# Autodesk Inventor assembly: AssemblyFullPrinter
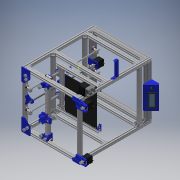
[picture p0: Inventor's stored thumbnail of the model, 180x180]
Saved by Autodesk Inventor 2018 (Build 220112000, 112)
## iProperties
Created: 2017-10-01
Part Number: AssemblyFullPrinter
Document SubType Name: Assembly
Designer: Jurjen
Author: Jurjen
## Documents named in this file (51)
- C:\Users\Jurjen\Documents\3D Printer\coreXY\Mechanical\AssemblyFullPrinter.iam
- C:\Users\Jurjen\Documents\3D Printer\coreXY\Mechanical\2020-350mm.ipt
- C:\Users\Jurjen\Documents\3D Printer\coreXY\Mechanical\2020-500mm.ipt
- C:\Users\Jurjen\Documents\3D Printer\coreXY\Mechanical\2020-corner-bracket.ipt
- C:\Users\Jurjen\Documents\3D Printer\coreXY\Mechanical\heated-bed.ipt
- C:\Users\Jurjen\Documents\3D Printer\coreXY\Mechanical\T8-lead-screw.ipt
- C:\Users\Jurjen\Documents\3D Printer\coreXY\Mechanical\motedis\GT2-Pulley-20-Teeth-5mm-Bore.ipt
- C:\Users\Jurjen\Documents\3D Printer\coreXY\Mechanical\motedis\Gt20.ipt
- C:\Users\Jurjen\Documents\3D Printer\coreXY\Mechanical\motedis\shaft-couple-flex.ipt
- C:\Users\Jurjen\Documents\3D Printer\coreXY\Mechanical\motedis\Motedis-SH8.ipt
- C:\Users\Jurjen\Documents\3D Printer\coreXY\Mechanical\rod-8mm.ipt
- C:\Users\Jurjen\Documents\3D Printer\coreXY\Mechanical\2020-290mm.ipt
- C:\Users\Jurjen\Documents\3D Printer\coreXY\Mechanical\2020-240mm.ipt
- C:\Users\Jurjen\Documents\3D Printer\coreXY\Mechanical\T8x2mm lead screw.ipt
- C:\Users\Jurjen\Documents\3D Printer\coreXY\Mechanical\OldhamCouplerBottom.ipt
- C:\Users\Jurjen\Documents\3D Printer\coreXY\Mechanical\OldhamCouplerMiddle.ipt
- C:\Users\Jurjen\Documents\3D Printer\coreXY\Mechanical\OldhamCouplerTop.ipt
- C:\Users\Jurjen\Documents\3D Printer\coreXY\Mechanical\M5-nut.ipt
- C:\Users\Jurjen\Documents\3D Printer\coreXY\Mechanical\bracket-GT2-left.ipt
- C:\Users\Jurjen\Documents\3D Printer\coreXY\Mechanical\M5x30mm.ipt
- C:\Users\Jurjen\Documents\3D Printer\coreXY\Mechanical\mount-heated-bed.ipt
- C:\Users\Jurjen\Documents\3D Printer\coreXY\Mechanical\bracket-GT2-right.ipt
- C:\Users\Jurjen\Documents\3D Printer\coreXY\Mechanical\spool-holder.ipt
- C:\Users\Jurjen\Documents\3D Printer\coreXY\Mechanical\nema-17.ipt
- C:\Users\Jurjen\Documents\3D Printer\coreXY\Mechanical\nema17-mount-left.ipt
- C:\Users\Jurjen\Documents\3D Printer\coreXY\Mechanical\nema17-mount-right.ipt
- C:\Users\Jurjen\Documents\3D Printer\coreXY\Mechanical\LMF8LUU.ipt
- C:\Users\Jurjen\Documents\3D Printer\coreXY\Mechanical\holder-LMF8LUU-z-axis.ipt
- C:\Users\Jurjen\Documents\3D Printer\coreXY\Mechanical\MGN-12-rail.ipt
- C:\Users\Jurjen\Documents\3D Printer\coreXY\Mechanical\2020-320mm.ipt
- C:\Users\Jurjen\Documents\3D Printer\coreXY\Mechanical\x-carriage-2020.ipt
- C:\Users\Jurjen\Documents\3D Printer\coreXY\Mechanical\X-connector-left.ipt
- C:\Users\Jurjen\Documents\3D Printer\coreXY\Mechanical\X-connector-right.ipt
- C:\Users\Jurjen\Documents\3D Printer\coreXY\Mechanical\MGN-12-H-carriage.ipt
- C:\Users\Jurjen\Documents\3D Printer\coreXY\Mechanical\ED3V6.ipt
- C:\Users\Jurjen\Documents\3D Printer\coreXY\Mechanical\x-carriage.ipt
- C:\Users\Jurjen\Documents\3D Printer\coreXY\Mechanical\x-carriage-holder.ipt
- C:\Users\Jurjen\Documents\3D Printer\coreXY\Mechanical\holder-GT2-x-carriage-left.ipt
- C:\Users\Jurjen\Documents\3D Printer\coreXY\Mechanical\M5x35mm-crosshead.ipt
- C:\Users\Jurjen\Documents\3D Printer\coreXY\Mechanical\extruder\e3d titan.iam
- C:\Users\Jurjen\Documents\3D Printer\coreXY\Mechanical\mount-extruder.ipt
- C:\Users\Jurjen\Documents\3D Printer\coreXY\Mechanical\NylonSpacerM5x5mm.ipt
- C:\Users\Jurjen\Documents\3D Printer\coreXY\Mechanical\holder-GT2-x-carriage-right.ipt
- C:\Users\Jurjen\Documents\3D Printer\coreXY\Mechanical\holder-bearing-z-axis.ipt
- C:\Users\Jurjen\Documents\3D Printer\coreXY\Mechanical\2040-350mm.ipt
- C:\Users\Jurjen\Documents\3D Printer\coreXY\Mechanical\nema17-mount-bottom-z-axis-v2.ipt
- C:\Users\Jurjen\Documents\3D Printer\coreXY\Mechanical\ramps-1.4 2004-LCD.ipt
- C:\Users\Jurjen\Documents\3D Printer\coreXY\Mechanical\holder-LCD-screen.ipt
- C:\Users\Jurjen\Documents\3D Printer\coreXY\Mechanical\spring-25mm.ipt
- C:\Users\Jurjen\Documents\3D Printer\coreXY\Mechanical\M3x40mm.ipt
- C:\Users\Jurjen\Documents\3D Printer\coreXY\Mechanical\2040-360mm.ipt
## Components (158 placed, 50 different names)
1. 2020-500mm:1 — Mate:1, Flush:2, Flush:14, Mate:85, Flush:37, Mate:90, Mate:92, Mate:93, Mate:94, Mate:131, Mate:132, Mate:163, Mate:165, Mate:166, Mate:168, Mate:287, Mate:288, Flush:54, Mate:359, Mate:360, Mate:434, Flush:78, Mate:459, Mate:471, Mate:472, Mate:473, Flush:92, Mate:552, Flush:107, Mate:573, Flush:112, Mate:584, Mate:595
2. 2020-500mm:2 — Mate:2, Flush:1, Flush:13, Flush:14, Mate:75, Mate:77, Mate:79, Mate:80, Mate:133, Mate:135, Mate:151, Mate:152, Mate:154, Mate:156, Mate:362, Mate:439, Mate:455, Mate:530, Flush:93, Mate:563, Flush:109, Flush:110, Flush:113, Mate:574, Mate:590, Mate:592
3. 2020-500mm:3 — Mate:8, Flush:12, Flush:13, Flush:15, Mate:82, Mate:83, Mate:86, Flush:39, Mate:136, Mate:138, Mate:149, Mate:150, Flush:67, Mate:367, Flush:82, Mate:456, Mate:501, Flush:85, Flush:86, Mate:516, Mate:517, Mate:522, Mate:523, Mate:562, Mate:585, Mate:591, Mate:593, Mate:594
4. 2020-500mm:4 — Mate:7, Flush:15, Flush:27, Mate:142, Mate:144, Mate:157, Mate:158, Mate:160, Mate:162, Mate:354, Flush:65, Mate:447, Mate:450, Mate:510, Mate:519, Mate:520, Mate:551, Flush:105, Mate:553, Flush:106, Mate:575, Flush:114, Mate:582, Mate:583, Mate:596
5. 2020-corner-bracket:38 — Mate:515, Mate:516, Mate:517
6. 2020-320mm:3 — Mate:353, Mate:354, Mate:355, Mate:356, Flush:65, Flush:66, Mate:357, Mate:358, Mate:368, Mate:369, Mate:373, Mate:374, Mate:388, Flush:73, Mate:446, Mate:448, Mate:460, Mate:461
7. 2020-320mm:4 — Flush:67, Mate:362, Mate:363, Mate:364, Flush:68, Mate:366, Flush:69, Mate:371, Mate:372, Mate:385, Mate:386, Mate:387, Flush:72, Mate:453, Mate:454, Mate:457, Mate:458
8. 2020-350mm:1 — Mate:1, Mate:2, Flush:1, Flush:2, Mate:19, Mate:23, Mate:76, Mate:95, Mate:294, Mate:303, Mate:304, Mate:307, Mate:308, Flush:66, Flush:68
9. 2020-350mm:4 — Mate:7, Mate:8, Flush:12, Mate:16, Mate:26, Flush:27, Mate:60, Mate:61, Mate:64, Mate:65, Mate:66, Mate:67, Mate:239, Mate:277, Mate:279, Flush:53, Mate:337, Flush:70, Mate:449, Mate:452, Mate:497, Mate:498, Mate:499, Mate:500, Flush:88, Flush:89, Mate:515
10. 2020-corner-bracket:1 — Mate:16, Mate:356, Mate:452
11. 2020-corner-bracket:2 — Mate:23, Mate:363, Mate:364
12. 2020-corner-bracket:3 — Mate:19, Mate:357, Mate:358
13. 2020-corner-bracket:4 — Mate:26, Mate:385, Mate:386
14. 2020-corner-bracket:10 — Mate:75, Mate:76, Mate:77
15. 2020-corner-bracket:13 — Mate:93, Mate:94, Mate:95, Mate:359
16. 2020-corner-bracket:33 — Mate:449, Mate:450
17. 2020-corner-bracket:34 — Mate:446, Mate:447, Mate:448
18. 2020-corner-bracket:35 — Mate:453, Mate:454, Mate:455
19. 2020-corner-bracket:36 — Mate:456, Mate:457, Mate:458
20. 2020-corner-bracket:37 — Mate:459, Mate:460, Mate:461
21. 2040-360mm:1 — Mate:552, Mate:553, Flush:106, Flush:107, Mate:554, Mate:555, Mate:558, Mate:559, Flush:108, Mate:572
22. 2040-360mm:2 — Mate:562, Mate:563, Flush:109, Flush:110, Mate:564, Mate:565, Mate:567, Flush:111, Mate:571
23. ramps-1.4 2004-LCD:1 — Flush:96, Mate:535, Mate:536
24. holder-LCD-screen:1 — Mate:534, Flush:95, Flush:96, Mate:535, Mate:536
25. 2040-350mm:1 — Mate:501, Flush:85, Flush:86, Mate:502, Mate:503, Mate:509, Flush:87, Mate:524, Mate:525
26. 2040-350mm:2 — Mate:526, Mate:527, Mate:528, Mate:529, Flush:92, Mate:530, Flush:93, Mate:534, Flush:95
27. 2020-corner-bracket:5 — Mate:503, Mate:559, Mate:560
28. 2020-corner-bracket:6 — Mate:502, Mate:570, Mate:571
29. 2020-corner-bracket:7 — Mate:528, Mate:567, Mate:569
30. 2020-corner-bracket:8 — Mate:529, Mate:558, Mate:561
31. 2020-corner-bracket:9 — Mate:79, Mate:80, Mate:526
32. 2020-corner-bracket:11 — Mate:82, Mate:83, Mate:565
33. 2020-corner-bracket:12 — Mate:90, Mate:92, Mate:527
34. 2020-corner-bracket:23 — Mate:151, Mate:152, Mate:564
35. 2020-corner-bracket:25 — Mate:157, Mate:158, Mate:555
36. 2020-corner-bracket:28 — Mate:166, Mate:168, Mate:554
37. 2020-350mm:10 — Mate:85, Flush:37, Mate:169, Mate:171, Mate:178, Mate:181, Flush:79, Mate:532, Mate:533
38. 2020-350mm:11 — Mate:86, Flush:39, Mate:174, Mate:176, Mate:179, Flush:80, Flush:81, Mate:518, Mate:521, Mate:599
39. 2020-320mm:5 — Mate:434, Mate:435, Flush:78, Flush:79, Flush:80, Mate:438, Mate:444, Mate:551, Flush:105, Mate:556, Mate:557, Mate:572
40. 2020-320mm:6 — Flush:81, Mate:439, Mate:441, Flush:82, Mate:443, Mate:566, Mate:568
41. 2020-corner-bracket:17 — Mate:133, Mate:135, Mate:532
42. 2020-corner-bracket:18 — Mate:131, Mate:132, Mate:533
43. 2020-corner-bracket:19 — Mate:136, Mate:138, Mate:524
44. 2020-corner-bracket:20 — Mate:142, Mate:144, Mate:525
45. 2020-corner-bracket:22 — Mate:149, Mate:150, Mate:568
46. 2020-corner-bracket:24 — Mate:154, Mate:156, Mate:566
47. 2020-corner-bracket:26 — Mate:160, Mate:162, Mate:557
48. 2020-corner-bracket:27 — Mate:163, Mate:165, Mate:556
49. 2020-corner-bracket:29 — Mate:169, Mate:178, Mate:441
50. 2020-corner-bracket:30 — Mate:171, Mate:181, Mate:435
51. 2020-corner-bracket:31 — Mate:174, Mate:438, Mate:444
52. 2020-corner-bracket:32 — Mate:176, Mate:179, Mate:443
53. 2020-corner-bracket:39 — Mate:521, Mate:522, Mate:523
54. 2020-corner-bracket:40 — Mate:518, Mate:519, Mate:520
55. 2020-corner-bracket:41 — Mate:548, Mate:549, Mate:550
56. 2020-corner-bracket:42 — Mate:545, Mate:546, Mate:547
57. spring-25mm:1 — Mate:537, Flush:98
58. spring-25mm:2 — Mate:538, Flush:100
59. spring-25mm:3 — Mate:539, Flush:97
60. spring-25mm:4 — Mate:540, Flush:99
61. 2020-corner-bracket:14 — Mate:122, Mate:123, Mate:124
62. 2020-corner-bracket:15 — Mate:119, Mate:120, Mate:121, Flush:49
63. nema17-mount-bottom-z-axis-v2:1 — Mate:506, Mate:507, Mate:508, Mate:509, Flush:87, Mate:510
64. holder-bearing-z-axis:1 — Mate:498, Mate:499, Mate:500, Mate:512, Flush:89, Mate:513
65. shaft-couple-flex:1 — Mate:59, Mate:114, Mate:293
66. LMF8LUU:1 — Mate:313, Mate:318, Mate:320, Mate:511
67. LMF8LUU:2 — Mate:314, Mate:324, Mate:326, Mate:327
68. holder-LMF8LUU-z-axis:1 — Mate:318, Mate:319, Mate:320, Mate:511, Angle:1, Flush:90
69. holder-LMF8LUU-z-axis:2 — Mate:324, Mate:326, Mate:327, Mate:328, Flush:91
70. T8-lead-screw:1 — Mate:59, Mate:114, Mate:115, Mate:116, Mate:117, Mate:118, Mate:315
71. nema-17:1 — Mate:293, Mate:315, Mate:506, Mate:507, Mate:508
72. rod-8mm:1 — Mate:73, Flush:34, Mate:314, Mate:505
73. rod-8mm:2 — Mate:74, Flush:35, Mate:313, Mate:504
74. heated-bed:1 — Mate:267, Mate:269, Mate:272, Mate:275, Mate:276, Mate:541, Flush:101, Flush:102, Mate:542, Mate:543, Flush:103, Flush:104, Mate:544
75. 2020-290mm:1 — Mate:109, Flush:45, Flush:46, Mate:123, Mate:265, Mate:266, Flush:52, Mate:270, Mate:271, Mate:545
76. 2020-290mm:2 — Mate:107, Flush:45, Flush:47, Mate:119, Flush:49, Mate:263, Mate:264, Flush:51, Mate:273, Mate:274, Mate:549
77. 2020-240mm:1 — Mate:103, Mate:104, Mate:105, Mate:107, Mate:109, Flush:46, Flush:47, Mate:110, Mate:120, Mate:121, Mate:122, Mate:124, Mate:319, Mate:328, Flush:88, Angle:1, Flush:90, Flush:91, Mate:546, Mate:547, Mate:548, Mate:550
78. mount-heated-bed:1 — Mate:263, Mate:264, Flush:51, Mate:267, Mate:276, Mate:537, Flush:98
79. mount-heated-bed:2 — Mate:265, Mate:266, Flush:52, Mate:269, Mate:538, Flush:100
80. mount-heated-bed:3 — Mate:270, Mate:271, Mate:272, Mate:540, Flush:99
81. mount-heated-bed:4 — Mate:273, Mate:274, Mate:275, Mate:539, Flush:97
82. M3x40mm:1 — Mate:541, Flush:101
83. M3x40mm:2 — Flush:102, Mate:542
84. M3x40mm:3 — Mate:543, Flush:103
85. M3x40mm:4 — Flush:104, Mate:544
86. Gt20:9 — Mate:486, Mate:488, Mate:489, Flush:83
87. Gt20:10 — Mate:485, Mate:496, Flush:84
88. NylonSpacerM5x5mm:3 — Mate:490, Mate:491
89. NylonSpacerM5x5mm:4 — Mate:487, Mate:489, Mate:491
90. M5-nut:9 — Mate:494, Mate:495
91. M5-nut:10 — Mate:492, Mate:493
92. M5x35mm-crosshead:3 — Mate:484, Mate:486, Mate:487, Mate:488, Mate:490, Mate:492
93. M5x35mm-crosshead:4 — Mate:483, Mate:485, Mate:494, Mate:496
94. holder-GT2-x-carriage-right:1 — Mate:480, Mate:481, Mate:482, Mate:483, Mate:484, Mate:493, Mate:495
95. NylonSpacerM5x5mm:2 — Mate:476, Mate:477
96. NylonSpacerM5x5mm:1 — Mate:474, Mate:475, Mate:477
97. Gt20:7 — Mate:424, Mate:433, Flush:76
98. Gt20:8 — Mate:423, Mate:427, Flush:77, Mate:475
99. MGN-12-rail:2 — Mate:373, Mate:374, Mate:388, Mate:394, Mate:395, Flush:73
100. MGN-12-rail:3 — Mate:371, Mate:372, Mate:387, Mate:392, Mate:393, Flush:72
101. MGN-12-H-carriage:1 — Mate:392, Mate:393, Mate:399, Mate:415
102. MGN-12-H-carriage:3 — Mate:394, Mate:395, Mate:396, Mate:397, Mate:398
103. GT2-Pulley-20-Teeth-5mm-Bore:2 — Mate:312, Flush:75, Flush:84
104. GT2-Pulley-20-Teeth-5mm-Bore:1 — Mate:297, Flush:56
105. bracket-GT2-right:1 — Mate:277, Mate:279, Mate:280, Mate:281, Mate:283, Mate:284, Mate:285, Mate:286, Flush:53, Mate:353, Mate:355
106. Gt20:5 — Mate:240, Mate:241, Flush:56, Mate:419, Flush:77
107. Gt20:6 — Mate:242, Mate:243, Mate:262, Flush:76
108. M5-nut:6 — Mate:260, Mate:283
109. bracket-GT2-left:1 — Mate:237, Mate:238, Mate:239, Mate:245, Mate:247, Mate:262, Mate:366, Mate:367, Flush:70, Mate:419
110. M5-nut:3 — Mate:244, Mate:245
111. M5-nut:5 — Mate:246, Mate:247
112. M5x30mm:1 — Mate:237, Mate:240, Mate:241, Mate:244
113. M5x30mm:2 — Mate:238, Mate:242, Mate:243, Mate:246
114. M5x30mm:3 — Mate:254, Mate:256, Mate:260, Mate:281
115. M5x30mm:4 — Mate:255, Mate:257, Mate:258, Mate:280
116. Gt20:2 — Mate:254, Mate:256, Mate:286, Flush:75
117. Gt20:4 — Mate:255, Mate:257, Mate:285, Flush:83
118. M5-nut:2 — Mate:258, Mate:284
119. nema-17:2 — Mate:297, Mate:298, Mate:299, Mate:300, Flush:57
120. nema-17:3 — Mate:309, Mate:310, Flush:58, Mate:311, Mate:312
121. nema17-mount-left:1 — Mate:294, Mate:298, Mate:299, Mate:300, Flush:57, Mate:303, Mate:304, Flush:69
122. nema17-mount-right:1 — Mate:307, Mate:308, Mate:309, Mate:310, Flush:58, Mate:311, Mate:360, Mate:368, Mate:369
123. spool-holder:1 — Mate:287, Mate:288, Flush:54
124. e3d titan:1 [sub-assembly] — Mate:465, Mate:466, Mate:470
125. mount-extruder:1 — Mate:465, Mate:466, Mate:467, Mate:468, Mate:469, Mate:470, Mate:471, Mate:472, Mate:473
126. nema-17:4 — Mate:467, Mate:468, Mate:469
127. 2020-320mm:7 — Mate:573, Flush:112, Flush:115, Mate:576, Mate:578, Mate:586
128. 2020-320mm:8 — Flush:113, Mate:574, Flush:116, Mate:579, Mate:580, Mate:588
129. 2020-350mm:12 — Mate:575, Flush:114, Flush:115, Flush:116, Mate:577, Mate:581, Mate:587, Mate:589, Mate:597, Mate:598, Mate:599
130. 2020-corner-bracket:43 — Mate:576, Mate:582
131. 2020-corner-bracket:44 — Mate:577, Mate:583, Mate:596
132. 2020-corner-bracket:45 — Mate:586, Mate:587, Mate:597
133. 2020-corner-bracket:46 — Mate:578, Mate:584, Mate:595
134. 2020-corner-bracket:47 — Mate:579, Mate:590, Mate:592
135. 2020-corner-bracket:48 — Mate:580, Mate:593, Mate:594
136. 2020-corner-bracket:49 — Mate:581, Mate:585, Mate:591
137. 2020-corner-bracket:50 — Mate:588, Mate:589, Mate:598
138. Motedis-SH8:1 — Flush:33, Mate:504
139. Motedis-SH8:2 — Flush:32, Mate:505
140. Motedis-SH8:3 — Mate:61, Mate:64, Mate:65, Flush:33, Mate:74, Flush:35, Mate:513
141. Motedis-SH8:4 — Mate:60, Mate:66, Mate:67, Flush:32, Mate:73, Flush:34, Mate:512
142. T8x2mm lead screw:1 — Mate:100, Mate:118
143. OldhamCouplerBottom:1 — Mate:99, Flush:43, Mate:100, Mate:117
144. OldhamCouplerMiddle:1 — Mate:99, Flush:43, Flush:44, Mate:102, Mate:115
145. OldhamCouplerTop:1 — Flush:44, Mate:102, Mate:103, Mate:104, Mate:105, Mate:110, Mate:116, Mate:337
146. MGN-12-rail:1 — Mate:381, Mate:389, Mate:390, Mate:391, Flush:71
147. x-carriage-2020:1 — Mate:377, Mate:381, Mate:384, Mate:389, Flush:71, Mate:409, Mate:410, Mate:411, Mate:421, Mate:422, Mate:432, Mate:480, Mate:481, Mate:482, Mate:497
148. X-connector-left:1 — Mate:377, Mate:396, Mate:397, Mate:398, Mate:410, Mate:411
149. X-connector-right:1 — Mate:384, Mate:399, Mate:409, Mate:415
150. MGN-12-H-carriage:2 — Mate:390, Mate:391, Mate:402, Mate:403, Mate:404
151. x-carriage-holder:1 — Mate:408, Mate:478, Mate:479
152. x-carriage:1 — Mate:402, Mate:403, Mate:404, Mate:405, Mate:408, Flush:74, Mate:478, Mate:479, Mate:514
153. holder-GT2-x-carriage-left:1 — Mate:421, Mate:422, Mate:425, Mate:426, Mate:429, Mate:431, Mate:432, Mate:514
154. M5-nut:7 — Mate:428, Mate:429
155. M5x35mm-crosshead:1 — Mate:423, Mate:426, Mate:427, Mate:428, Mate:474, Mate:476
156. M5-nut:8 — Mate:430, Mate:431
157. M5x35mm-crosshead:2 — Mate:424, Mate:425, Mate:430, Mate:433
158. ED3V6:1 — Mate:405, Flush:74
## Relationships (440: Mate 362, Flush 77, Angle 1)
- Mate:1: 2020-500mm:1 ↔ 2020-350mm:1
- Mate:2: 2020-500mm:2 ↔ 2020-350mm:1
- Flush:1: 2020-500mm:2 ↔ 2020-350mm:1
- Flush:2: 2020-500mm:1 ↔ 2020-350mm:1
- Mate:7: 2020-500mm:4 ↔ 2020-350mm:4
- Mate:8: 2020-500mm:3 ↔ 2020-350mm:4
- Flush:12: 2020-500mm:3 ↔ 2020-350mm:4
- Flush:13: 2020-500mm:2 ↔ 2020-500mm:3
- Flush:14: 2020-500mm:1 ↔ 2020-500mm:2
- Flush:15: 2020-500mm:3 ↔ 2020-500mm:4
- Mate:16: 2020-350mm:4 ↔ 2020-corner-bracket:1
- Mate:19: 2020-350mm:1 ↔ 2020-corner-bracket:3
- Mate:23: 2020-350mm:1 ↔ 2020-corner-bracket:2
- Mate:26: 2020-350mm:4 ↔ 2020-corner-bracket:4
- Flush:27: 2020-500mm:4 ↔ 2020-350mm:4
- Mate:59 (-8 mm): shaft-couple-flex:1 ↔ T8-lead-screw:1
- Mate:60: 2020-350mm:4 ↔ Motedis-SH8:4
- Mate:61: 2020-350mm:4 ↔ Motedis-SH8:3
- Mate:64: 2020-350mm:4 ↔ Motedis-SH8:3
- Mate:65: 2020-350mm:4 ↔ Motedis-SH8:3
- Mate:66: 2020-350mm:4 ↔ Motedis-SH8:4
- Mate:67: 2020-350mm:4 ↔ Motedis-SH8:4
- Flush:32: Motedis-SH8:2 ↔ Motedis-SH8:4
- Flush:33: Motedis-SH8:1 ↔ Motedis-SH8:3
- Mate:73: rod-8mm:1 ↔ Motedis-SH8:4
- Mate:74: rod-8mm:2 ↔ Motedis-SH8:3
- Flush:34 (-5 mm): rod-8mm:1 ↔ Motedis-SH8:4
- Flush:35 (-5 mm): rod-8mm:2 ↔ Motedis-SH8:3
- Mate:75: 2020-500mm:2 ↔ 2020-corner-bracket:10
- Mate:76: 2020-350mm:1 ↔ 2020-corner-bracket:10
- Mate:77: 2020-500mm:2 ↔ 2020-corner-bracket:10
- Mate:79: 2020-500mm:2 ↔ 2020-corner-bracket:9
- Mate:80: 2020-500mm:2 ↔ 2020-corner-bracket:9
- Mate:82: 2020-500mm:3 ↔ 2020-corner-bracket:11
- Mate:83: 2020-500mm:3 ↔ 2020-corner-bracket:11
- Mate:85: 2020-500mm:1 ↔ 2020-350mm:10
- Flush:37: 2020-500mm:1 ↔ 2020-350mm:10
- Mate:86: 2020-500mm:3 ↔ 2020-350mm:11
- Flush:39: 2020-500mm:3 ↔ 2020-350mm:11
- Mate:90: 2020-500mm:1 ↔ 2020-corner-bracket:12
- Mate:92: 2020-500mm:1 ↔ 2020-corner-bracket:12
- Mate:93: 2020-500mm:1 ↔ 2020-corner-bracket:13
- Mate:94: 2020-500mm:1 ↔ 2020-corner-bracket:13
- Mate:95: 2020-350mm:1 ↔ 2020-corner-bracket:13
- Mate:99: OldhamCouplerBottom:1 ↔ OldhamCouplerMiddle:1
- Flush:43: OldhamCouplerBottom:1 ↔ OldhamCouplerMiddle:1
- Mate:100: T8x2mm lead screw:1 ↔ OldhamCouplerBottom:1
- Flush:44: OldhamCouplerMiddle:1 ↔ OldhamCouplerTop:1
- Mate:102: OldhamCouplerMiddle:1 ↔ OldhamCouplerTop:1
- Mate:103: 2020-240mm:1 ↔ OldhamCouplerTop:1
- Mate:104: 2020-240mm:1 ↔ OldhamCouplerTop:1
- Mate:105: 2020-240mm:1 ↔ OldhamCouplerTop:1
- Mate:107: 2020-290mm:2 ↔ 2020-240mm:1
- Mate:109: 2020-290mm:1 ↔ 2020-240mm:1
- Flush:45: 2020-290mm:1 ↔ 2020-290mm:2
- Flush:46: 2020-290mm:1 ↔ 2020-240mm:1
- Flush:47: 2020-290mm:2 ↔ 2020-240mm:1
- Mate:110: 2020-240mm:1 ↔ OldhamCouplerTop:1
- Mate:114: shaft-couple-flex:1 ↔ T8-lead-screw:1
- Mate:115: T8-lead-screw:1 ↔ OldhamCouplerMiddle:1
- Mate:116: T8-lead-screw:1 ↔ OldhamCouplerTop:1
- Mate:117: T8-lead-screw:1 ↔ OldhamCouplerBottom:1
- Mate:118: T8-lead-screw:1 ↔ T8x2mm lead screw:1
- Mate:119: 2020-corner-bracket:15 ↔ 2020-290mm:2
- Mate:120: 2020-corner-bracket:15 ↔ 2020-240mm:1
- Mate:121: 2020-corner-bracket:15 ↔ 2020-240mm:1
- Flush:49: 2020-corner-bracket:15 ↔ 2020-290mm:2
- Mate:122: 2020-corner-bracket:14 ↔ 2020-240mm:1
- Mate:123: 2020-corner-bracket:14 ↔ 2020-290mm:1
- Mate:124: 2020-corner-bracket:14 ↔ 2020-240mm:1
- Mate:131: 2020-500mm:1 ↔ 2020-corner-bracket:18
- Mate:132: 2020-500mm:1 ↔ 2020-corner-bracket:18
- Mate:133: 2020-500mm:2 ↔ 2020-corner-bracket:17
- Mate:135: 2020-500mm:2 ↔ 2020-corner-bracket:17
- Mate:136: 2020-500mm:3 ↔ 2020-corner-bracket:19
- Mate:138: 2020-500mm:3 ↔ 2020-corner-bracket:19
- Mate:142: 2020-500mm:4 ↔ 2020-corner-bracket:20
- Mate:144: 2020-500mm:4 ↔ 2020-corner-bracket:20
- Mate:149: 2020-500mm:3 ↔ 2020-corner-bracket:22
- Mate:150: 2020-500mm:3 ↔ 2020-corner-bracket:22
- Mate:151: 2020-500mm:2 ↔ 2020-corner-bracket:23
- Mate:152: 2020-500mm:2 ↔ 2020-corner-bracket:23
- Mate:154: 2020-500mm:2 ↔ 2020-corner-bracket:24
- Mate:156: 2020-500mm:2 ↔ 2020-corner-bracket:24
- Mate:157: 2020-500mm:4 ↔ 2020-corner-bracket:25
- Mate:158: 2020-500mm:4 ↔ 2020-corner-bracket:25
- Mate:160: 2020-500mm:4 ↔ 2020-corner-bracket:26
- Mate:162: 2020-500mm:4 ↔ 2020-corner-bracket:26
- Mate:163: 2020-500mm:1 ↔ 2020-corner-bracket:27
- Mate:165: 2020-500mm:1 ↔ 2020-corner-bracket:27
- Mate:166: 2020-500mm:1 ↔ 2020-corner-bracket:28
- Mate:168: 2020-500mm:1 ↔ 2020-corner-bracket:28
- Mate:169: 2020-350mm:10 ↔ 2020-corner-bracket:29
- Mate:171: 2020-350mm:10 ↔ 2020-corner-bracket:30
- Mate:174: 2020-350mm:11 ↔ 2020-corner-bracket:31
- Mate:176: 2020-350mm:11 ↔ 2020-corner-bracket:32
- Mate:178: 2020-350mm:10 ↔ 2020-corner-bracket:29
- Mate:179: 2020-350mm:11 ↔ 2020-corner-bracket:32
- Mate:181: 2020-350mm:10 ↔ 2020-corner-bracket:30
- Mate:237: bracket-GT2-left:1 ↔ M5x30mm:1
- Mate:238: bracket-GT2-left:1 ↔ M5x30mm:2
- Mate:239: 2020-350mm:4 ↔ bracket-GT2-left:1
- Mate:240: Gt20:5 ↔ M5x30mm:1
- Mate:241: Gt20:5 ↔ M5x30mm:1
- Mate:242: Gt20:6 ↔ M5x30mm:2
- Mate:243: Gt20:6 ↔ M5x30mm:2
- Mate:244: M5-nut:3 ↔ M5x30mm:1
- Mate:245: bracket-GT2-left:1 ↔ M5-nut:3
- Mate:246: M5-nut:5 ↔ M5x30mm:2
- Mate:247: bracket-GT2-left:1 ↔ M5-nut:5
- Mate:254: M5x30mm:3 ↔ Gt20:2
- Mate:255: M5x30mm:4 ↔ Gt20:4
- Mate:256: M5x30mm:3 ↔ Gt20:2
- Mate:257: M5x30mm:4 ↔ Gt20:4
- Mate:258: M5x30mm:4 ↔ M5-nut:2
- Mate:260: M5-nut:6 ↔ M5x30mm:3
- Mate:262: Gt20:6 ↔ bracket-GT2-left:1
- Mate:263: 2020-290mm:2 ↔ mount-heated-bed:1
- Mate:264: 2020-290mm:2 ↔ mount-heated-bed:1
- Flush:51: 2020-290mm:2 ↔ mount-heated-bed:1
- Mate:265: 2020-290mm:1 ↔ mount-heated-bed:2
- Mate:266: 2020-290mm:1 ↔ mount-heated-bed:2
- Flush:52: 2020-290mm:1 ↔ mount-heated-bed:2
- Mate:267: heated-bed:1 ↔ mount-heated-bed:1
- Mate:269: heated-bed:1 ↔ mount-heated-bed:2
- Mate:270: 2020-290mm:1 ↔ mount-heated-bed:3
- Mate:271: 2020-290mm:1 ↔ mount-heated-bed:3
- Mate:272: heated-bed:1 ↔ mount-heated-bed:3
- Mate:273: 2020-290mm:2 ↔ mount-heated-bed:4
- Mate:274: 2020-290mm:2 ↔ mount-heated-bed:4
- Mate:275: heated-bed:1 ↔ mount-heated-bed:4
- Mate:276 (25 mm): heated-bed:1 ↔ mount-heated-bed:1
- Mate:277: 2020-350mm:4 ↔ bracket-GT2-right:1
- Mate:279: 2020-350mm:4 ↔ bracket-GT2-right:1
- Mate:280: bracket-GT2-right:1 ↔ M5x30mm:4
- Mate:281: bracket-GT2-right:1 ↔ M5x30mm:3
- Mate:283: bracket-GT2-right:1 ↔ M5-nut:6
- Mate:284: bracket-GT2-right:1 ↔ M5-nut:2
- Mate:285: bracket-GT2-right:1 ↔ Gt20:4
- Mate:286: bracket-GT2-right:1 ↔ Gt20:2
- Flush:53: 2020-350mm:4 ↔ bracket-GT2-right:1
- Mate:287: 2020-500mm:1 ↔ spool-holder:1
- Mate:288: 2020-500mm:1 ↔ spool-holder:1
- Flush:54: 2020-500mm:1 ↔ spool-holder:1
- Mate:293 (-8 mm): shaft-couple-flex:1 ↔ nema-17:1
- Mate:294: 2020-350mm:1 ↔ nema17-mount-left:1
- Mate:297: GT2-Pulley-20-Teeth-5mm-Bore:1 ↔ nema-17:2
- Flush:56: GT2-Pulley-20-Teeth-5mm-Bore:1 ↔ Gt20:5
- Mate:298: nema-17:2 ↔ nema17-mount-left:1
- Mate:299: nema-17:2 ↔ nema17-mount-left:1
- Mate:300: nema-17:2 ↔ nema17-mount-left:1
- Flush:57: nema-17:2 ↔ nema17-mount-left:1
- Mate:303: 2020-350mm:1 ↔ nema17-mount-left:1
- Mate:304: 2020-350mm:1 ↔ nema17-mount-left:1
- Mate:307: 2020-350mm:1 ↔ nema17-mount-right:1
- Mate:308: 2020-350mm:1 ↔ nema17-mount-right:1
- Mate:309: nema-17:3 ↔ nema17-mount-right:1
- Mate:310: nema-17:3 ↔ nema17-mount-right:1
- Flush:58: nema-17:3 ↔ nema17-mount-right:1
- Mate:311: nema-17:3 ↔ nema17-mount-right:1
- Mate:312: GT2-Pulley-20-Teeth-5mm-Bore:2 ↔ nema-17:3
- Mate:313: LMF8LUU:1 ↔ rod-8mm:2
- Mate:314: LMF8LUU:2 ↔ rod-8mm:1
- Mate:315: T8-lead-screw:1 ↔ nema-17:1
- Mate:318: LMF8LUU:1 ↔ holder-LMF8LUU-z-axis:1
- Mate:319: holder-LMF8LUU-z-axis:1 ↔ 2020-240mm:1
- Mate:320: LMF8LUU:1 ↔ holder-LMF8LUU-z-axis:1
- Mate:324: LMF8LUU:2 ↔ holder-LMF8LUU-z-axis:2
- Mate:326: LMF8LUU:2 ↔ holder-LMF8LUU-z-axis:2
- Mate:327: LMF8LUU:2 ↔ holder-LMF8LUU-z-axis:2
- Mate:328: holder-LMF8LUU-z-axis:2 ↔ 2020-240mm:1
- Mate:337: 2020-350mm:4 ↔ OldhamCouplerTop:1
- Mate:353: 2020-320mm:3 ↔ bracket-GT2-right:1
- Mate:354: 2020-500mm:4 ↔ 2020-320mm:3
- Mate:355: 2020-320mm:3 ↔ bracket-GT2-right:1
- Mate:356: 2020-320mm:3 ↔ 2020-corner-bracket:1
- Flush:65: 2020-500mm:4 ↔ 2020-320mm:3
- Flush:66: 2020-320mm:3 ↔ 2020-350mm:1
- Mate:357: 2020-320mm:3 ↔ 2020-corner-bracket:3
- Mate:358: 2020-320mm:3 ↔ 2020-corner-bracket:3
- Mate:359: 2020-500mm:1 ↔ 2020-corner-bracket:13
- Mate:360: 2020-500mm:1 ↔ nema17-mount-right:1
- Flush:67: 2020-500mm:3 ↔ 2020-320mm:4
- Mate:362: 2020-500mm:2 ↔ 2020-320mm:4
- Mate:363: 2020-320mm:4 ↔ 2020-corner-bracket:2
- Mate:364: 2020-320mm:4 ↔ 2020-corner-bracket:2
- Flush:68: 2020-320mm:4 ↔ 2020-350mm:1
- Mate:366: 2020-320mm:4 ↔ bracket-GT2-left:1
- Mate:367: 2020-500mm:3 ↔ bracket-GT2-left:1
- Mate:368: 2020-320mm:3 ↔ nema17-mount-right:1
- Mate:369: 2020-320mm:3 ↔ nema17-mount-right:1
- Flush:69: 2020-320mm:4 ↔ nema17-mount-left:1
- Mate:371: 2020-320mm:4 ↔ MGN-12-rail:3
- Mate:372: 2020-320mm:4 ↔ MGN-12-rail:3
- Mate:373: 2020-320mm:3 ↔ MGN-12-rail:2
- Mate:374: 2020-320mm:3 ↔ MGN-12-rail:2
- Flush:70: 2020-350mm:4 ↔ bracket-GT2-left:1
- Mate:377: x-carriage-2020:1 ↔ X-connector-left:1
- Mate:381: MGN-12-rail:1 ↔ x-carriage-2020:1
- Mate:384: x-carriage-2020:1 ↔ X-connector-right:1
- Mate:385: 2020-320mm:4 ↔ 2020-corner-bracket:4
- Mate:386: 2020-320mm:4 ↔ 2020-corner-bracket:4
- Mate:387: 2020-320mm:4 ↔ MGN-12-rail:3
- Mate:388: 2020-320mm:3 ↔ MGN-12-rail:2
- Mate:389: MGN-12-rail:1 ↔ x-carriage-2020:1
- Mate:390: MGN-12-rail:1 ↔ MGN-12-H-carriage:2
- Mate:391: MGN-12-rail:1 ↔ MGN-12-H-carriage:2
- Mate:392: MGN-12-rail:3 ↔ MGN-12-H-carriage:1
- Mate:393: MGN-12-rail:3 ↔ MGN-12-H-carriage:1
- Mate:394: MGN-12-rail:2 ↔ MGN-12-H-carriage:3
- Mate:395: MGN-12-rail:2 ↔ MGN-12-H-carriage:3
- Mate:396: MGN-12-H-carriage:3 ↔ X-connector-left:1
- Mate:397: MGN-12-H-carriage:3 ↔ X-connector-left:1
- Mate:398: MGN-12-H-carriage:3 ↔ X-connector-left:1
- Mate:399: MGN-12-H-carriage:1 ↔ X-connector-right:1
- Flush:71: MGN-12-rail:1 ↔ x-carriage-2020:1
- Flush:72: 2020-320mm:4 ↔ MGN-12-rail:3
- Flush:73: 2020-320mm:3 ↔ MGN-12-rail:2
- Mate:402: MGN-12-H-carriage:2 ↔ x-carriage:1
- Mate:403: MGN-12-H-carriage:2 ↔ x-carriage:1
- Mate:404: MGN-12-H-carriage:2 ↔ x-carriage:1
- Mate:405: x-carriage:1 ↔ ED3V6:1
- Mate:408: x-carriage-holder:1 ↔ x-carriage:1
- Flush:74: x-carriage:1 ↔ ED3V6:1
- Flush:75: GT2-Pulley-20-Teeth-5mm-Bore:2 ↔ Gt20:2
- Mate:409: x-carriage-2020:1 ↔ X-connector-right:1
- Mate:410: x-carriage-2020:1 ↔ X-connector-left:1
- Mate:411 (-25 mm): x-carriage-2020:1 ↔ X-connector-left:1
- Mate:415: MGN-12-H-carriage:1 ↔ X-connector-right:1
- Mate:419: Gt20:5 ↔ bracket-GT2-left:1
- Mate:421: x-carriage-2020:1 ↔ holder-GT2-x-carriage-left:1
- Mate:422: x-carriage-2020:1 ↔ holder-GT2-x-carriage-left:1
- Mate:423: Gt20:8 ↔ M5x35mm-crosshead:1
- Mate:424: Gt20:7 ↔ M5x35mm-crosshead:2
- Mate:425: holder-GT2-x-carriage-left:1 ↔ M5x35mm-crosshead:2
- Mate:426: holder-GT2-x-carriage-left:1 ↔ M5x35mm-crosshead:1
- Mate:427: Gt20:8 ↔ M5x35mm-crosshead:1
- Mate:428: M5-nut:7 ↔ M5x35mm-crosshead:1
- Mate:429: holder-GT2-x-carriage-left:1 ↔ M5-nut:7
- Mate:430: M5-nut:8 ↔ M5x35mm-crosshead:2
- Mate:431: holder-GT2-x-carriage-left:1 ↔ M5-nut:8
- Mate:432: x-carriage-2020:1 ↔ holder-GT2-x-carriage-left:1
- Mate:433: Gt20:7 ↔ M5x35mm-crosshead:2
- Flush:76: Gt20:7 ↔ Gt20:6
- Flush:77: Gt20:8 ↔ Gt20:5
- Mate:434: 2020-500mm:1 ↔ 2020-320mm:5
- Mate:435: 2020-320mm:5 ↔ 2020-corner-bracket:30
- Flush:78: 2020-500mm:1 ↔ 2020-320mm:5
- Flush:79: 2020-350mm:10 ↔ 2020-320mm:5
- Flush:80: 2020-350mm:11 ↔ 2020-320mm:5
- Flush:81: 2020-350mm:11 ↔ 2020-320mm:6
- Mate:438: 2020-320mm:5 ↔ 2020-corner-bracket:31
- Mate:439: 2020-500mm:2 ↔ 2020-320mm:6
- Mate:441: 2020-320mm:6 ↔ 2020-corner-bracket:29
- Flush:82: 2020-500mm:3 ↔ 2020-320mm:6
- Mate:443: 2020-320mm:6 ↔ 2020-corner-bracket:32
- Mate:444: 2020-320mm:5 ↔ 2020-corner-bracket:31
- Mate:446: 2020-320mm:3 ↔ 2020-corner-bracket:34
- Mate:447: 2020-500mm:4 ↔ 2020-corner-bracket:34
- Mate:448: 2020-320mm:3 ↔ 2020-corner-bracket:34
- Mate:449: 2020-350mm:4 ↔ 2020-corner-bracket:33
- Mate:450: 2020-500mm:4 ↔ 2020-corner-bracket:33
- Mate:452: 2020-350mm:4 ↔ 2020-corner-bracket:1
- Mate:453: 2020-320mm:4 ↔ 2020-corner-bracket:35
- Mate:454: 2020-320mm:4 ↔ 2020-corner-bracket:35
- Mate:455: 2020-500mm:2 ↔ 2020-corner-bracket:35
- Mate:456: 2020-500mm:3 ↔ 2020-corner-bracket:36
- Mate:457: 2020-320mm:4 ↔ 2020-corner-bracket:36
- Mate:458: 2020-320mm:4 ↔ 2020-corner-bracket:36
- Mate:459: 2020-500mm:1 ↔ 2020-corner-bracket:37
- Mate:460: 2020-320mm:3 ↔ 2020-corner-bracket:37
- Mate:461: 2020-320mm:3 ↔ 2020-corner-bracket:37
- Mate:465: e3d titan:1 ↔ mount-extruder:1
- Mate:466: e3d titan:1 ↔ mount-extruder:1
- Mate:467: mount-extruder:1 ↔ nema-17:4
- Mate:468: mount-extruder:1 ↔ nema-17:4
- Mate:469: mount-extruder:1 ↔ nema-17:4
- Mate:470: e3d titan:1 ↔ mount-extruder:1
- Mate:471: 2020-500mm:1 ↔ mount-extruder:1
- Mate:472: 2020-500mm:1 ↔ mount-extruder:1
- Mate:473: 2020-500mm:1 ↔ mount-extruder:1
- Mate:474: NylonSpacerM5x5mm:1 ↔ M5x35mm-crosshead:1
- Mate:475: NylonSpacerM5x5mm:1 ↔ Gt20:8
- Mate:476: NylonSpacerM5x5mm:2 ↔ M5x35mm-crosshead:1
- Mate:477: NylonSpacerM5x5mm:2 ↔ NylonSpacerM5x5mm:1
- Mate:478: x-carriage-holder:1 ↔ x-carriage:1
- Mate:479: x-carriage-holder:1 ↔ x-carriage:1
- Mate:480: holder-GT2-x-carriage-right:1 ↔ x-carriage-2020:1
- Mate:481: holder-GT2-x-carriage-right:1 ↔ x-carriage-2020:1
- Mate:482: holder-GT2-x-carriage-right:1 ↔ x-carriage-2020:1
- Mate:483: M5x35mm-crosshead:4 ↔ holder-GT2-x-carriage-right:1
- Mate:484: M5x35mm-crosshead:3 ↔ holder-GT2-x-carriage-right:1
- Mate:485: Gt20:10 ↔ M5x35mm-crosshead:4
- Mate:486: Gt20:9 ↔ M5x35mm-crosshead:3
- Mate:487: NylonSpacerM5x5mm:4 ↔ M5x35mm-crosshead:3
- Mate:488: Gt20:9 ↔ M5x35mm-crosshead:3
- Mate:489: Gt20:9 ↔ NylonSpacerM5x5mm:4
- Mate:490: NylonSpacerM5x5mm:3 ↔ M5x35mm-crosshead:3
- Mate:491: NylonSpacerM5x5mm:3 ↔ NylonSpacerM5x5mm:4
- Mate:492: M5-nut:10 ↔ M5x35mm-crosshead:3
- Mate:493: M5-nut:10 ↔ holder-GT2-x-carriage-right:1
- Flush:83: Gt20:9 ↔ Gt20:4
- Mate:494: M5-nut:9 ↔ M5x35mm-crosshead:4
- Mate:495: M5-nut:9 ↔ holder-GT2-x-carriage-right:1
- Mate:496: Gt20:10 ↔ M5x35mm-crosshead:4
- Flush:84: Gt20:10 ↔ GT2-Pulley-20-Teeth-5mm-Bore:2
- Mate:497: 2020-350mm:4 ↔ x-carriage-2020:1
- Mate:498: 2020-350mm:4 ↔ holder-bearing-z-axis:1
- Mate:499: 2020-350mm:4 ↔ holder-bearing-z-axis:1
- Mate:500: 2020-350mm:4 ↔ holder-bearing-z-axis:1
- Mate:501: 2020-500mm:3 ↔ 2040-350mm:1
- Flush:85: 2020-500mm:3 ↔ 2040-350mm:1
- Flush:86: 2020-500mm:3 ↔ 2040-350mm:1
- Mate:502: 2040-350mm:1 ↔ 2020-corner-bracket:6
- Mate:503: 2040-350mm:1 ↔ 2020-corner-bracket:5
- Mate:504: rod-8mm:2 ↔ Motedis-SH8:1
- Mate:505: rod-8mm:1 ↔ Motedis-SH8:2
- Mate:506: nema17-mount-bottom-z-axis-v2:1 ↔ nema-17:1
- Mate:507: nema17-mount-bottom-z-axis-v2:1 ↔ nema-17:1
- Mate:508: nema17-mount-bottom-z-axis-v2:1 ↔ nema-17:1
- Mate:509: 2040-350mm:1 ↔ nema17-mount-bottom-z-axis-v2:1
- Flush:87: 2040-350mm:1 ↔ nema17-mount-bottom-z-axis-v2:1
- Mate:510 (155 mm): 2020-500mm:4 ↔ nema17-mount-bottom-z-axis-v2:1
- Flush:88: 2020-350mm:4 ↔ 2020-240mm:1
- Mate:511: LMF8LUU:1 ↔ holder-LMF8LUU-z-axis:1
- Mate:512 (20 mm): holder-bearing-z-axis:1 ↔ Motedis-SH8:4
- Flush:89: 2020-350mm:4 ↔ holder-bearing-z-axis:1
- Mate:513 (20 mm): holder-bearing-z-axis:1 ↔ Motedis-SH8:3
- Angle:1 (0 deg): holder-LMF8LUU-z-axis:1 ↔ 2020-240mm:1
- Flush:90: holder-LMF8LUU-z-axis:1 ↔ 2020-240mm:1
- Flush:91: holder-LMF8LUU-z-axis:2 ↔ 2020-240mm:1
- Mate:514: x-carriage:1 ↔ holder-GT2-x-carriage-left:1
- Mate:515: 2020-corner-bracket:38 ↔ 2020-350mm:4
- Mate:516: 2020-500mm:3 ↔ 2020-corner-bracket:38
- Mate:517: 2020-500mm:3 ↔ 2020-corner-bracket:38
- Mate:518: 2020-350mm:11 ↔ 2020-corner-bracket:40
- Mate:519: 2020-500mm:4 ↔ 2020-corner-bracket:40
- Mate:520: 2020-500mm:4 ↔ 2020-corner-bracket:40
- Mate:521: 2020-350mm:11 ↔ 2020-corner-bracket:39
- Mate:522: 2020-500mm:3 ↔ 2020-corner-bracket:39
- Mate:523: 2020-500mm:3 ↔ 2020-corner-bracket:39
- Mate:524: 2040-350mm:1 ↔ 2020-corner-bracket:19
- Mate:525: 2040-350mm:1 ↔ 2020-corner-bracket:20
- Mate:526: 2040-350mm:2 ↔ 2020-corner-bracket:9
- Mate:527: 2040-350mm:2 ↔ 2020-corner-bracket:12
- Mate:528: 2040-350mm:2 ↔ 2020-corner-bracket:7
- Mate:529: 2040-350mm:2 ↔ 2020-corner-bracket:8
- Flush:92: 2020-500mm:1 ↔ 2040-350mm:2
- Mate:530: 2020-500mm:2 ↔ 2040-350mm:2
- Flush:93: 2020-500mm:2 ↔ 2040-350mm:2
- Mate:532: 2020-350mm:10 ↔ 2020-corner-bracket:17
- Mate:533: 2020-350mm:10 ↔ 2020-corner-bracket:18
- Mate:534: holder-LCD-screen:1 ↔ 2040-350mm:2
- Flush:95: holder-LCD-screen:1 ↔ 2040-350mm:2
- Flush:96 (-2 mm): ramps-1.4 2004-LCD:1 ↔ holder-LCD-screen:1
- Mate:535: ramps-1.4 2004-LCD:1 ↔ holder-LCD-screen:1
- Mate:536: ramps-1.4 2004-LCD:1 ↔ holder-LCD-screen:1
- Mate:537: spring-25mm:1 ↔ mount-heated-bed:1
- Mate:538: spring-25mm:2 ↔ mount-heated-bed:2
- Mate:539: spring-25mm:3 ↔ mount-heated-bed:4
- Flush:97: spring-25mm:3 ↔ mount-heated-bed:4
- Flush:98: spring-25mm:1 ↔ mount-heated-bed:1
- Mate:540: spring-25mm:4 ↔ mount-heated-bed:3
- Flush:99: spring-25mm:4 ↔ mount-heated-bed:3
- Flush:100: spring-25mm:2 ↔ mount-heated-bed:2
- Mate:541: heated-bed:1 ↔ M3x40mm:1
- Flush:101: heated-bed:1 ↔ M3x40mm:1
- Flush:102: heated-bed:1 ↔ M3x40mm:2
- Mate:542: heated-bed:1 ↔ M3x40mm:2
- Mate:543: heated-bed:1 ↔ M3x40mm:3
- Flush:103: heated-bed:1 ↔ M3x40mm:3
- Flush:104: heated-bed:1 ↔ M3x40mm:4
- Mate:544: heated-bed:1 ↔ M3x40mm:4
- Mate:545: 2020-corner-bracket:42 ↔ 2020-290mm:1
- Mate:546: 2020-corner-bracket:42 ↔ 2020-240mm:1
- Mate:547: 2020-corner-bracket:42 ↔ 2020-240mm:1
- Mate:548: 2020-corner-bracket:41 ↔ 2020-240mm:1
- Mate:549: 2020-corner-bracket:41 ↔ 2020-290mm:2
- Mate:550: 2020-corner-bracket:41 ↔ 2020-240mm:1
- Mate:551: 2020-500mm:4 ↔ 2020-320mm:5
- Flush:105: 2020-500mm:4 ↔ 2020-320mm:5
- Mate:552: 2020-500mm:1 ↔ 2040-360mm:1
- Mate:553: 2020-500mm:4 ↔ 2040-360mm:1
- Flush:106: 2020-500mm:4 ↔ 2040-360mm:1
- Flush:107: 2020-500mm:1 ↔ 2040-360mm:1
- Mate:554: 2040-360mm:1 ↔ 2020-corner-bracket:28
- Mate:555: 2040-360mm:1 ↔ 2020-corner-bracket:25
- Mate:556: 2020-320mm:5 ↔ 2020-corner-bracket:27
- Mate:557: 2020-320mm:5 ↔ 2020-corner-bracket:26
- Mate:558: 2040-360mm:1 ↔ 2020-corner-bracket:8
- Mate:559: 2040-360mm:1 ↔ 2020-corner-bracket:5
- Flush:108 (-10 mm): 2040-360mm:1
- Mate:560: 2020-corner-bracket:5
- Mate:561: 2020-corner-bracket:8
- Mate:562: 2020-500mm:3 ↔ 2040-360mm:2
- Mate:563: 2020-500mm:2 ↔ 2040-360mm:2
- Flush:109: 2020-500mm:2 ↔ 2040-360mm:2
- Flush:110: 2020-500mm:2 ↔ 2040-360mm:2
- Mate:564: 2040-360mm:2 ↔ 2020-corner-bracket:23
- Mate:565: 2040-360mm:2 ↔ 2020-corner-bracket:11
- Mate:566: 2020-320mm:6 ↔ 2020-corner-bracket:24
- Mate:567: 2040-360mm:2 ↔ 2020-corner-bracket:7
- Mate:568: 2020-320mm:6 ↔ 2020-corner-bracket:22
- Flush:111 (-10 mm): 2040-360mm:2
- Mate:569: 2020-corner-bracket:7
- Mate:570: 2020-corner-bracket:6
- Mate:571: 2040-360mm:2 ↔ 2020-corner-bracket:6
- Mate:572 (25 mm): 2040-360mm:1 ↔ 2020-320mm:5
- Mate:573: 2020-500mm:1 ↔ 2020-320mm:7
- Flush:112: 2020-500mm:1 ↔ 2020-320mm:7
- Flush:113: 2020-500mm:2 ↔ 2020-320mm:8
- Mate:574: 2020-500mm:2 ↔ 2020-320mm:8
- Mate:575: 2020-500mm:4 ↔ 2020-350mm:12
- Flush:114: 2020-500mm:4 ↔ 2020-350mm:12
- Flush:115: 2020-320mm:7 ↔ 2020-350mm:12
- Flush:116: 2020-320mm:8 ↔ 2020-350mm:12
- Mate:576: 2020-320mm:7 ↔ 2020-corner-bracket:43
- Mate:577: 2020-350mm:12 ↔ 2020-corner-bracket:44
- Mate:578: 2020-320mm:7 ↔ 2020-corner-bracket:46
- Mate:579: 2020-320mm:8 ↔ 2020-corner-bracket:47
- Mate:580: 2020-320mm:8 ↔ 2020-corner-bracket:48
- Mate:581: 2020-350mm:12 ↔ 2020-corner-bracket:49
- Mate:582: 2020-500mm:4 ↔ 2020-corner-bracket:43
- Mate:583: 2020-500mm:4 ↔ 2020-corner-bracket:44
- Mate:584: 2020-500mm:1 ↔ 2020-corner-bracket:46
- Mate:585: 2020-500mm:3 ↔ 2020-corner-bracket:49
- Mate:586: 2020-320mm:7 ↔ 2020-corner-bracket:45
- Mate:587: 2020-350mm:12 ↔ 2020-corner-bracket:45
- Mate:588: 2020-320mm:8 ↔ 2020-corner-bracket:50
- Mate:589: 2020-350mm:12 ↔ 2020-corner-bracket:50
- Mate:590: 2020-500mm:2 ↔ 2020-corner-bracket:47
- Mate:591: 2020-500mm:3 ↔ 2020-corner-bracket:49
- Mate:592: 2020-500mm:2 ↔ 2020-corner-bracket:47
- Mate:593: 2020-500mm:3 ↔ 2020-corner-bracket:48
- Mate:594: 2020-500mm:3 ↔ 2020-corner-bracket:48
- Mate:595: 2020-500mm:1 ↔ 2020-corner-bracket:46
- Mate:596: 2020-500mm:4 ↔ 2020-corner-bracket:44
- Mate:597: 2020-350mm:12 ↔ 2020-corner-bracket:45
- Mate:598: 2020-350mm:12 ↔ 2020-corner-bracket:50
- Mate:599 (200 mm): 2020-350mm:11 ↔ 2020-350mm:12
